# Autodesk Inventor assembly: Drivetrain V1
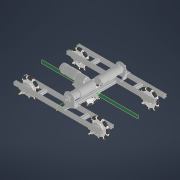
[picture p0: Inventor's stored thumbnail of the model, 180x180]
Saved by Autodesk Inventor 2022 (Build 260153000, 153)
## iProperties
Created: 2021-12-01
Part Number: Drivetrain V1
Document SubType Name: Assembly
Designer: izack
Author: izack
## Documents named in this file (13)
- D:\Robotics\ComputerAidedDesign\2021-22\FTC\#12456 Big Red\Drivetrain\Omni Wheel Drive\Drivetrain V1.iam
- D:\Robotics\ComputerAidedDesign\2021-22\FTC\#12456 Big Red\Drivetrain\Omni Wheel Drive\15mm Extrusion - 420mm - 90° Ends.ipt
- D:\Robotics\ComputerAidedDesign\2021-22\FTC\#12456 Big Red\Drivetrain\Omni Wheel Drive\15mm Extrusion - 7.5in - 90 Ends.ipt
- D:\Robotics\ComputerAidedDesign\2021-22\FTC\#12456 Big Red\Drivetrain\Omni Wheel Drive\15mm Extrusion - 34.4mm - 90° Ends.ipt
- D:\Robotics\ComputerAidedDesign\2021-22\FTC\#12456 Big Red\Drivetrain\Omni Wheel Drive\omni wheels-26 tooth sproket.iam
- D:\Robotics\ComputerAidedDesign\2021-22\FTC\#12456 Big Red\Drivetrain\Omni Wheel Drive\Gobilda 1620 motor mount with motor.iam
- D:\Robotics\ComputerAidedDesign\2021-22\FTC\#13822 Robovikes\Proof of Concept\13in^3 drivetrain parts\5202 Series Yellow Jacket Planetary Gear Motor.ipt
- D:\Robotics\ComputerAidedDesign\2021-22\FTC\#12456 Big Red\Drivetrain\Omni Wheel Drive\5202 Series Yellow Jacket planetary Gear Small Motor Mount.ipt
- D:\Robotics\ComputerAidedDesign\2021-22\FTC\#13822 Robovikes\Proof of Concept\13in^3 drivetrain parts\10 Tooth #25 D-Shaft Sprocket - 4 Pack.ipt
- D:\Robotics\ComputerAidedDesign\2021-22\FTC\#12456 Big Red\Drivetrain\Omni Wheel Drive\Custom Gears\Design Accelerator\Spur Gear12.ipt
- D:\Robotics\ComputerAidedDesign\2021-22\FTC\#12456 Big Red\Drivetrain\Omni Wheel Drive\Custom Gears\Design Accelerator\Spur Gear21.ipt
- D:\Robotics\ComputerAidedDesign\2021-22\FTC\#12456 Big Red\Drivetrain\Omni Wheel Drive\Custom Gears\Design Accelerator\Spur Gear13.ipt
- D:\Robotics\ComputerAidedDesign\2021-22\FTC\#12456 Big Red\Drivetrain\Omni Wheel Drive\Custom Gears\Design Accelerator\Spur Gear22.ipt
## Components (27 placed, 10 different names)
1. 15mm Extrusion - 420mm - 90° Ends:1 — Mate:1, Flush:1, Flush:5, Mate:3, Mate:11, Mate:12, Symmetry:3, Flush:46
2. 15mm Extrusion - 420mm - 90° Ends:2 — Flush:1, Flush:2, Flush:5, Flush:6, Mate:3, Mate:4, Mate:7, Mate:8, Flush:9, Flush:10, Flush:13, Flush:14, Mate:16, Mate:18, Mate:26, Flush:17, Flush:47
3. 15mm Extrusion - 420mm - 90° Ends:3 — Flush:2, Flush:3, Flush:4, Flush:6, Mate:2, Mate:4, Flush:7, Flush:8, Mate:9, Mate:10, Flush:11, Flush:12, Flush:15, Mate:13, Flush:16, Mate:22, Symmetry:2, Flush:43, Mate:46
4. 15mm Extrusion - 420mm - 90° Ends:4 — Flush:3, Flush:4, Mate:2, Mate:5, Mate:6, Mate:14, Mate:15, Mate:17, Symmetry:2, Symmetry:3, Flush:44, Flush:45
5. 15mm Extrusion - 7.5in - 90 Ends:1 — Mate:9, Flush:11, Mate:19, Symmetry:1
6. 15mm Extrusion - 7.5in - 90 Ends:2 — Mate:10, Flush:12, Mate:19, Mate:20, Mate:21, Symmetry:1, Mate:39, Flush:18
7. 15mm Extrusion - 34.4mm - 90° Ends:1 — Mate:6, Flush:8, Flush:45
8. 15mm Extrusion - 34.4mm - 90° Ends:2 — Mate:5, Flush:7, Flush:44
9. 15mm Extrusion - 34.4mm - 90° Ends:3 — Mate:8, Flush:10, Flush:47
10. 15mm Extrusion - 34.4mm - 90° Ends:4 — Mate:7, Flush:9, Flush:46
11. omni wheels-26 tooth sproket:1 [sub-assembly] — Mate:14, Flush:16, Mate:17
12. omni wheels-26 tooth sproket:2 [sub-assembly] — Flush:13, Mate:11, Mate:18
13. omni wheels-26 tooth sproket:3 [sub-assembly] — Mate:12, Flush:14, Mate:16
14. omni wheels-26 tooth sproket:4 [sub-assembly] — Flush:15, Mate:13, Mate:15
15. Gobilda 1620 motor mount with motor:1 [sub-assembly] — Mate:20, Mate:21, Mate:22, Mate:23, Mate:24, Mate:25
16. 5202 Series Yellow Jacket Planetary Gear Motor:1 — Mate:23, Mate:24, Mate:25, Mate:42, Mate:54, Mate:55
17. 5202 Series Yellow Jacket planetary Gear Small Motor Mount:1 — Mate:26, Flush:17, Mate:27, Mate:28, Mate:29, Mate:47
18. 5202 Series Yellow Jacket Planetary Gear Motor:2 — Mate:27, Mate:28, Mate:29, Mate:37, Mate:38
19. 5202 Series Yellow Jacket Planetary Gear Motor:3 — Mate:49, Mate:50, Mate:51, Mate:52, Mate:53
20. 10 Tooth #25 D-Shaft Sprocket - 4 Pack:1 — Mate:37, Mate:38
21. omni wheels-26 tooth sproket:5 [sub-assembly] — Mate:39, Flush:18, Mate:40, Mate:43, Mate:44, Mate:45, Mate:56, Mate:57
22. Spur Gear1:1 — Flush:42, Mate:42
23. Spur Gear2:1 — Mate:43, Mate:44, Mate:45, Flush:42
24. 5202 Series Yellow Jacket planetary Gear Small Motor Mount:2 — Flush:43, Mate:46, Mate:48, Mate:49, Mate:50, Mate:51
25. 10 Tooth #25 D-Shaft Sprocket - 4 Pack:2 — Mate:52, Mate:53
26. Spur Gear1:2 — Mate:54, Mate:55
27. Spur Gear2:2 — Mate:56, Mate:57
## Relationships (77: Mate 50, Flush 24, Symmetry 3)
- Mate:1: 15mm Extrusion - 420mm - 90° Ends:1
- Flush:1: 15mm Extrusion - 420mm - 90° Ends:1 ↔ 15mm Extrusion - 420mm - 90° Ends:2
- Flush:2: 15mm Extrusion - 420mm - 90° Ends:2 ↔ 15mm Extrusion - 420mm - 90° Ends:3
- Flush:3: 15mm Extrusion - 420mm - 90° Ends:3 ↔ 15mm Extrusion - 420mm - 90° Ends:4
- Flush:4: 15mm Extrusion - 420mm - 90° Ends:3 ↔ 15mm Extrusion - 420mm - 90° Ends:4
- Flush:5: 15mm Extrusion - 420mm - 90° Ends:1 ↔ 15mm Extrusion - 420mm - 90° Ends:2
- Flush:6: 15mm Extrusion - 420mm - 90° Ends:2 ↔ 15mm Extrusion - 420mm - 90° Ends:3
- Mate:2 (34.4 mm): 15mm Extrusion - 420mm - 90° Ends:3 ↔ 15mm Extrusion - 420mm - 90° Ends:4
- Mate:3 (34.4 mm): 15mm Extrusion - 420mm - 90° Ends:1 ↔ 15mm Extrusion - 420mm - 90° Ends:2
- Mate:4 (190.5 mm): 15mm Extrusion - 420mm - 90° Ends:2 ↔ 15mm Extrusion - 420mm - 90° Ends:3
- Mate:5: 15mm Extrusion - 420mm - 90° Ends:4 ↔ 15mm Extrusion - 34.4mm - 90° Ends:2
- Mate:6: 15mm Extrusion - 420mm - 90° Ends:4 ↔ 15mm Extrusion - 34.4mm - 90° Ends:1
- Mate:7: 15mm Extrusion - 420mm - 90° Ends:2 ↔ 15mm Extrusion - 34.4mm - 90° Ends:4
- Mate:8: 15mm Extrusion - 420mm - 90° Ends:2 ↔ 15mm Extrusion - 34.4mm - 90° Ends:3
- Flush:7: 15mm Extrusion - 420mm - 90° Ends:3 ↔ 15mm Extrusion - 34.4mm - 90° Ends:2
- Flush:8: 15mm Extrusion - 420mm - 90° Ends:3 ↔ 15mm Extrusion - 34.4mm - 90° Ends:1
- Flush:9: 15mm Extrusion - 420mm - 90° Ends:2 ↔ 15mm Extrusion - 34.4mm - 90° Ends:4
- Flush:10: 15mm Extrusion - 420mm - 90° Ends:2 ↔ 15mm Extrusion - 34.4mm - 90° Ends:3
- Mate:9: 15mm Extrusion - 420mm - 90° Ends:3 ↔ 15mm Extrusion - 7.5in - 90 Ends:1
- Mate:10: 15mm Extrusion - 420mm - 90° Ends:3 ↔ 15mm Extrusion - 7.5in - 90 Ends:2
- Flush:11: 15mm Extrusion - 420mm - 90° Ends:3 ↔ 15mm Extrusion - 7.5in - 90 Ends:1
- Flush:12: 15mm Extrusion - 420mm - 90° Ends:3 ↔ 15mm Extrusion - 7.5in - 90 Ends:2
- Flush:13: 15mm Extrusion - 420mm - 90° Ends:2 ↔ omni wheels-26 tooth sproket:2
- Mate:11: 15mm Extrusion - 420mm - 90° Ends:1 ↔ omni wheels-26 tooth sproket:2
- Mate:12: 15mm Extrusion - 420mm - 90° Ends:1 ↔ omni wheels-26 tooth sproket:3
- Flush:14: 15mm Extrusion - 420mm - 90° Ends:2 ↔ omni wheels-26 tooth sproket:3
- Flush:15: 15mm Extrusion - 420mm - 90° Ends:3 ↔ omni wheels-26 tooth sproket:4
- Mate:13: 15mm Extrusion - 420mm - 90° Ends:3 ↔ omni wheels-26 tooth sproket:4
- Mate:14: 15mm Extrusion - 420mm - 90° Ends:4 ↔ omni wheels-26 tooth sproket:1
- Flush:16: 15mm Extrusion - 420mm - 90° Ends:3 ↔ omni wheels-26 tooth sproket:1
- Mate:15 (-25 mm): 15mm Extrusion - 420mm - 90° Ends:4 ↔ omni wheels-26 tooth sproket:4
- Mate:16 (-25 mm): 15mm Extrusion - 420mm - 90° Ends:2 ↔ omni wheels-26 tooth sproket:3
- Mate:17 (-25 mm): 15mm Extrusion - 420mm - 90° Ends:4 ↔ omni wheels-26 tooth sproket:1
- Mate:18 (-25 mm): 15mm Extrusion - 420mm - 90° Ends:2 ↔ omni wheels-26 tooth sproket:2
- Mate:19 (34.4 mm): 15mm Extrusion - 7.5in - 90 Ends:1 ↔ 15mm Extrusion - 7.5in - 90 Ends:2
- Mate:20: 15mm Extrusion - 7.5in - 90 Ends:2 ↔ Gobilda 1620 motor mount with motor:1
- Mate:21: 15mm Extrusion - 7.5in - 90 Ends:2 ↔ Gobilda 1620 motor mount with motor:1
- Mate:22 (63.25 mm): 15mm Extrusion - 420mm - 90° Ends:3 ↔ Gobilda 1620 motor mount with motor:1
- Mate:23: Gobilda 1620 motor mount with motor:1 ↔ 5202 Series Yellow Jacket Planetary Gear Motor:1
- Mate:24: Gobilda 1620 motor mount with motor:1 ↔ 5202 Series Yellow Jacket Planetary Gear Motor:1
- Mate:25: Gobilda 1620 motor mount with motor:1 ↔ 5202 Series Yellow Jacket Planetary Gear Motor:1
- Mate:26: 15mm Extrusion - 420mm - 90° Ends:2 ↔ 5202 Series Yellow Jacket planetary Gear Small Motor Mount:1
- Flush:17: 15mm Extrusion - 420mm - 90° Ends:2 ↔ 5202 Series Yellow Jacket planetary Gear Small Motor Mount:1
- Mate:27: 5202 Series Yellow Jacket planetary Gear Small Motor Mount:1 ↔ 5202 Series Yellow Jacket Planetary Gear Motor:2
- Mate:28: 5202 Series Yellow Jacket planetary Gear Small Motor Mount:1 ↔ 5202 Series Yellow Jacket Planetary Gear Motor:2
- Mate:29: 5202 Series Yellow Jacket planetary Gear Small Motor Mount:1 ↔ 5202 Series Yellow Jacket Planetary Gear Motor:2
- Symmetry:1: 15mm Extrusion - 7.5in - 90 Ends:1 ↔ 15mm Extrusion - 7.5in - 90 Ends:2
- Symmetry:2: 15mm Extrusion - 420mm - 90° Ends:3 ↔ 15mm Extrusion - 420mm - 90° Ends:4
- Mate:35
- Mate:37: 5202 Series Yellow Jacket Planetary Gear Motor:2 ↔ 10 Tooth #25 D-Shaft Sprocket - 4 Pack:1
- Mate:38 (1 mm): 5202 Series Yellow Jacket Planetary Gear Motor:2 ↔ 10 Tooth #25 D-Shaft Sprocket - 4 Pack:1
- Mate:39: 15mm Extrusion - 7.5in - 90 Ends:2 ↔ omni wheels-26 tooth sproket:5
- Flush:18: 15mm Extrusion - 7.5in - 90 Ends:2 ↔ omni wheels-26 tooth sproket:5
- Symmetry:3: 15mm Extrusion - 420mm - 90° Ends:1 ↔ 15mm Extrusion - 420mm - 90° Ends:4
- Mate:40 (-18 mm): omni wheels-26 tooth sproket:5
- Flush:42: Spur Gear1:1 ↔ Spur Gear2:1
- Mate:42: 5202 Series Yellow Jacket Planetary Gear Motor:1 ↔ Spur Gear1:1
- Mate:43: omni wheels-26 tooth sproket:5 ↔ Spur Gear2:1
- Mate:44: omni wheels-26 tooth sproket:5 ↔ Spur Gear2:1
- Mate:45: omni wheels-26 tooth sproket:5 ↔ Spur Gear2:1
- Flush:43: 15mm Extrusion - 420mm - 90° Ends:3 ↔ 5202 Series Yellow Jacket planetary Gear Small Motor Mount:2
- Mate:46: 15mm Extrusion - 420mm - 90° Ends:3 ↔ 5202 Series Yellow Jacket planetary Gear Small Motor Mount:2
- Mate:47: 5202 Series Yellow Jacket planetary Gear Small Motor Mount:1
- Mate:48: 5202 Series Yellow Jacket planetary Gear Small Motor Mount:2
- Mate:49: 5202 Series Yellow Jacket Planetary Gear Motor:3 ↔ 5202 Series Yellow Jacket planetary Gear Small Motor Mount:2
- Mate:50: 5202 Series Yellow Jacket Planetary Gear Motor:3 ↔ 5202 Series Yellow Jacket planetary Gear Small Motor Mount:2
- Mate:51: 5202 Series Yellow Jacket Planetary Gear Motor:3 ↔ 5202 Series Yellow Jacket planetary Gear Small Motor Mount:2
- Flush:44 (100 mm): 15mm Extrusion - 420mm - 90° Ends:4 ↔ 15mm Extrusion - 34.4mm - 90° Ends:2
- Flush:45 (100 mm): 15mm Extrusion - 420mm - 90° Ends:4 ↔ 15mm Extrusion - 34.4mm - 90° Ends:1
- Flush:46 (100 mm): 15mm Extrusion - 420mm - 90° Ends:1 ↔ 15mm Extrusion - 34.4mm - 90° Ends:4
- Flush:47 (100 mm): 15mm Extrusion - 420mm - 90° Ends:2 ↔ 15mm Extrusion - 34.4mm - 90° Ends:3
- Mate:52: 5202 Series Yellow Jacket Planetary Gear Motor:3 ↔ 10 Tooth #25 D-Shaft Sprocket - 4 Pack:2
- Mate:53 (6 mm): 5202 Series Yellow Jacket Planetary Gear Motor:3 ↔ 10 Tooth #25 D-Shaft Sprocket - 4 Pack:2
- Mate:54: 5202 Series Yellow Jacket Planetary Gear Motor:1 ↔ Spur Gear1:2
- Mate:55 (5 mm): 5202 Series Yellow Jacket Planetary Gear Motor:1 ↔ Spur Gear1:2
- Mate:56: omni wheels-26 tooth sproket:5 ↔ Spur Gear2:2
- Mate:57: omni wheels-26 tooth sproket:5 ↔ Spur Gear2:2
